# Autodesk Inventor assembly: sensing part
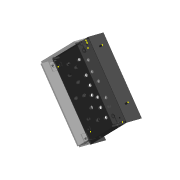
[picture p0: Inventor's stored thumbnail of the model, 180x180]
Saved by Autodesk Inventor 2019 (Build 230136000, 136)
## iProperties
Part Number: sensing part
Document SubType Name: Assembly
Designer: Ranjita
Author: Ranjita
## Documents named in this file (4)
- D:\mechanical tutorial\sensing part.iam
- C:\Users\Ranjita\Documents\Inventor\Content Center Files\R2019\base2.ipt
- C:\Users\Ranjita\Documents\Inventor\Content Center Files\R2019\mooootoooor.ipt
- C:\Users\Ranjita\Documents\Inventor\Content Center Files\R2019\transparent base.ipt
## Components (6 placed, 3 different names)
1. base2:1 — Rotational:1, Rotational:2, Rotational:3, Rotational:4, Rigid:1
2. mooootoooor:1 — Rotational:1
3. mooootoooor:2 — Rotational:2
4. mooootoooor:3 — Rotational:4
5. mooootoooor:4 — Rotational:3
6. transparent base:1 — Rigid:1
## Relationships (5: RevoluteJoint 4, WeldJoint 1)
- Rotational:1 [RevoluteJoint]: base2:1 ↔ mooootoooor:1
- Rotational:2 [RevoluteJoint]: base2:1 ↔ mooootoooor:2
- Rotational:3 [RevoluteJoint]: base2:1 ↔ mooootoooor:4
- Rotational:4 [RevoluteJoint]: base2:1 ↔ mooootoooor:3
- Rigid:1 [WeldJoint]: base2:1 ↔ transparent base:1
